# Autodesk Inventor assembly: Carrello semplice
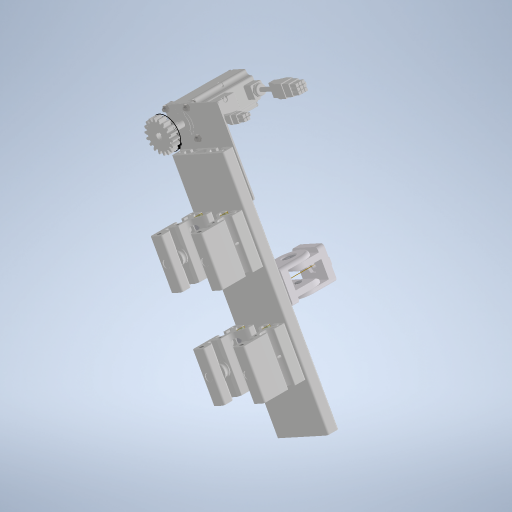
[picture p0: Inventor's stored thumbnail of the model, 512x512]
Saved by Autodesk Inventor 2023 (Build 270158000, 158)
## iProperties
Created: 2021-12-30
Part Number: Carrello semplice
Document SubType Name: Assembly
Designer: matte
Author: matte
## Documents named in this file (9)
- C:\Users\matte\Documents\GitHub\MDM-CyberOrto-CAD\Pezzi singoli\Supporto lineare\Carrello semplice.iam
- C:\Users\matte\Documents\GitHub\MDM-CyberOrto-CAD\Pezzi singoli\Supporto lineare\Piastra-supporto.ipt
- C:\Users\matte\Documents\GitHub\MDM-CyberOrto-CAD\Parker components\08-Linear Application\06-Linear Roller System\01-Roller System 6\30-401.ipt
- C:\Users\matte\Documents\GitHub\MDM-CyberOrto-CAD\Pezzi singoli\Supporto lineare\Doppia Giuntura.iam
- C:\Users\matte\Documents\GitHub\MDM-CyberOrto-CAD\Parker components\05-Handles_Hinges\13-Pivot Joints\23-010.iam
- C:\Users\matte\Documents\GitHub\MDM-CyberOrto-CAD\Parker components\02-Fasteners\10-Standard T-Nuts\20-058.ipt
- C:\Users\matte\Documents\GitHub\MDM-CyberOrto-CAD\Parker components\02-Fasteners\16-Screws\01-Metric Screws\01-Button Head\24-116-8.ipt
- C:\Users\matte\Documents\GitHub\MDM-CyberOrto-CAD\Parker components\02-Fasteners\10-Standard T-Nuts\20-050.ipt
- C:\Users\matte\Documents\GitHub\MDM-CyberOrto-CAD\Rack_Pinion\Motor_assembly.iam
## Components (15 placed, 8 different names)
1. Piastra-supporto:1 — Allineato:7, Coincidente:6, Coincidente:7, Coincidente:11, Coincidente:12, Allineato:20, Allineato:21, Angolo:1, Coincidente:21, Coincidente:24, Allineato:26, Coincidente:69, Coincidente:70
2. 30-401:1 — Coincidente:19, Coincidente:56
3. 30-401:2 — Coincidente:24
4. 30-401:3 — Coincidente:68
5. 30-401:4 — Coincidente:8
6. 23-010:1 [sub-assembly] — Allineato:20, Allineato:21, Coincidente:19, Coincidente:20, Coincidente:22, Coincidente:23
7. 20-058:1 — Coincidente:20, Angolo:1, Coincidente:21
8. 24-116-8:1 — Coincidente:22, Coincidente:23
9. 20-050:1 — Coincidente:56
10. 20-050:2 — Coincidente:68
11. Motor_assembly:1 [sub-assembly] — Allineato:26, Coincidente:69, Coincidente:70
12. Doppia Giuntura:2 [sub-assembly] — Coincidente:11, Coincidente:12, Coincidente:15
13. Doppia Giuntura:1 [sub-assembly] — Coincidente:6, Coincidente:7, Coincidente:8, Coincidente:15
14. Doppia Giuntura:3 [sub-assembly]
15. Doppia Giuntura:4 [sub-assembly]
## Component patterns: (2 elements, first: Doppia Giuntura:2 + Doppia Giuntura:1)
## Relationships (32: Mate 21, Flush 10, Angle 1)
- [Mate]: Piastra-supporto:1 ↔ 30-401:1
- [Flush]: Piastra-supporto:1 ↔ 30-401:1
- [Flush]: Piastra-supporto:1 ↔ 30-401:2
- [Mate]: Piastra-supporto:1 ↔ 30-401:2
- [Mate] (60 mm): 30-401:1 ↔ 30-401:2
- [Mate]: Piastra-supporto:1 ↔ 30-401:3
- [Flush]: Piastra-supporto:1 ↔ 30-401:3
- [Flush]: 30-401:1 ↔ 30-401:3
- [Mate]: Piastra-supporto:1 ↔ 30-401:4
- [Flush]: Piastra-supporto:1 ↔ 30-401:4
- [Flush]: 30-401:2 ↔ 30-401:4
- Allineato:7 [Flush]: Piastra-supporto:1
- Coincidente:6 [Mate]: Piastra-supporto:1 ↔ Doppia Giuntura:1
- Coincidente:7 [Mate]: Piastra-supporto:1 ↔ Doppia Giuntura:1
- Coincidente:8 [Mate]: 30-401:4 ↔ Doppia Giuntura:1
- Coincidente:11 [Mate]: Piastra-supporto:1 ↔ Doppia Giuntura:2
- Coincidente:12 [Mate]: Piastra-supporto:1 ↔ Doppia Giuntura:2
- Coincidente:15 [Mate]: Doppia Giuntura:2 ↔ Doppia Giuntura:1
- Allineato:20 [Flush]: Piastra-supporto:1 ↔ 23-010:1
- Allineato:21 [Flush]: Piastra-supporto:1 ↔ 23-010:1
- Coincidente:19 [Mate] (30 mm): 30-401:1 ↔ 23-010:1
- Coincidente:20 [Mate]: 23-010:1 ↔ 20-058:1
- Angolo:1 [Angle] (0 deg): Piastra-supporto:1 ↔ 20-058:1
- Coincidente:21 [Mate]: Piastra-supporto:1 ↔ 20-058:1
- Coincidente:22 [Mate]: 23-010:1 ↔ 24-116-8:1
- Coincidente:23 [Mate]: 23-010:1 ↔ 24-116-8:1
- Coincidente:24 [Mate] (60 mm): Piastra-supporto:1 ↔ 30-401:2
- Coincidente:56 [Mate]: 30-401:1 ↔ 20-050:1
- Coincidente:68 [Mate]: 30-401:3 ↔ 20-050:2
- Allineato:26 [Flush]: Piastra-supporto:1 ↔ Motor_assembly:1
- Coincidente:69 [Mate]: Piastra-supporto:1 ↔ Motor_assembly:1
- Coincidente:70 [Mate] (10 mm): Piastra-supporto:1 ↔ Motor_assembly:1
